# Autodesk Inventor assembly: Wheel
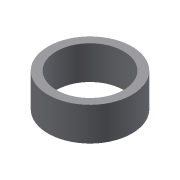
[picture p0: Inventor's stored thumbnail of the model, 180x180]
Saved by Autodesk Inventor 2017 (Build 210142000, 142)
## iProperties
Created: 2017-03-11
Part Number: Wheel
Document SubType Name: Assembly
Designer: zallen
Author: zallen
## Documents named in this file (3)
- C:\Users\zallen\Documents\Autodesk Inventor Projects\LaundryRobot_v0.1\Wheel.iam
- C:\Users\zallen\Documents\Autodesk Inventor Projects\LaundryRobot_v0.1\Wheel.ipt
- C:\Users\zallen\Documents\Autodesk Inventor Projects\Robot Maid I\Tire.ipt
## Components (2 placed, 2 different names)
1. Wheel:1 — Flush:1, Mate:1
2. Tire:1 — Flush:1, Mate:1
## Relationships (2: Flush 1, Mate 1)
- Flush:1: Wheel:1 ↔ Tire:1
- Mate:1: Wheel:1 ↔ Tire:1
